# Autodesk Inventor assembly: am 42 Tooth Pully with Bearings
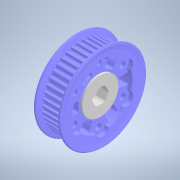
[picture p0: Inventor's stored thumbnail of the model, 180x180]
Saved by Autodesk Inventor 2021 (Build 250183000, 183)
## iProperties
Created: 2021-03-03
Part Number: am 42 Tooth Pully with Bearings
Document SubType Name: Assembly
Designer: aidan
Author: aidan
## Documents named in this file (3)
- C:\Users\aidan\Desktop\T3 Robotics\CAD\Generic and Stock\am 42 Tooth Pully with Bearings.iam
- C:\Users\aidan\Desktop\T3 Robotics\CAD\Generic and Stock\am 42 Tooth Pulley Full Shrinkwrap.ipt
- C:\Users\aidan\Desktop\T3 Robotics\CAD\Bearing  for THUNDER.ipt
## Components (3 placed, 2 different names)
1. am 42 Tooth Pulley Full Shrinkwrap:1 — Insert:1, Insert:2
2. Bearing  for THUNDER:1 — Flush:1, Flush:2, Insert:1
3. Bearing  for THUNDER:2 — Flush:1, Flush:2, Insert:2
## Relationships (4: Flush 2, Insert 2)
- Flush:1: Bearing  for THUNDER:1 ↔ Bearing  for THUNDER:2
- Flush:2: Bearing  for THUNDER:1 ↔ Bearing  for THUNDER:2
- Insert:1: am 42 Tooth Pulley Full Shrinkwrap:1 ↔ Bearing  for THUNDER:1
- Insert:2: am 42 Tooth Pulley Full Shrinkwrap:1 ↔ Bearing  for THUNDER:2
